# Autodesk Inventor assembly: Ensamble tensor + eje
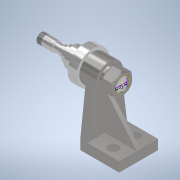
[picture p0: Inventor's stored thumbnail of the model, 180x180]
Saved by Autodesk Inventor 2021 (Build 250183000, 183)
## iProperties
Created: 2021-01-10
Part Number: Ensamble tensor + eje
Document SubType Name: Assembly
Designer: dieku
Author: dieku
## Documents named in this file (5)
- C:\Users\dieku\Documents\GitHub\tallerDibujoIngenieria\Ensambles\Ensamble tensor + eje.iam
- C:\Users\dieku\Documents\GitHub\tallerDibujoIngenieria\Partes\Soporte_Tensor.ipt
- C:\Users\dieku\Documents\Inventor\Content Center Files\R2021\en-US\DIN 934\DIN 934 - M27 x 3.ipt
- C:\Users\dieku\Documents\Inventor\Content Center Files\R2021\en-US\DIN 127 - W\DIN 127 - A 27.ipt
- C:\Users\dieku\Documents\GitHub\tallerDibujoIngenieria\Partes\Eje\Eje Final.iam
## Components (4 placed, 4 different names)
1. Soporte_Tensor:1 — Angle:1, Mate:1, Mate:2, Insert:1
2. DIN 934 - replaced by DIN EN 24032/28673/28674 M27:1 — Mate:3
3. DIN 127 - withdrawn A 27:1 — Insert:1, Mate:3
4. Eje Final:1 [sub-assembly] — Angle:1, Mate:1, Mate:2
## Relationships (5: Mate 3, Angle 1, Insert 1)
- Angle:1 (180 deg): Soporte_Tensor:1 ↔ Eje Final:1
- Mate:1: Soporte_Tensor:1 ↔ Eje Final:1
- Mate:2: Soporte_Tensor:1 ↔ Eje Final:1
- Insert:1: Soporte_Tensor:1 ↔ DIN 127 - withdrawn A 27:1
- Mate:3: DIN 934 - replaced by DIN EN 24032/28673/28674 M27:1 ↔ DIN 127 - withdrawn A 27:1
